# Autodesk Inventor assembly: unterArm
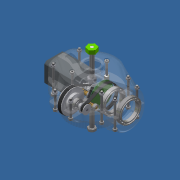
[picture p0: Inventor's stored thumbnail of the model, 180x180]
Saved by Autodesk Inventor 2016 (Build 200138000, 138)
## iProperties
Created: 2015-08-25
Part Number: unterArm
Material: Generisch
Document SubType Name: Assembly
Designer: 4ndreas
Mass: 1359.16 g
Surface Area: 1900.72 cm^2
Volume: 704.74 cm^3
Density: 1.92859 g/cm^3
Author: 4ndreas
## Documents named in this file (26)
- C:\Users\4ndreas\Documents\Inventor\RobotARM v2\v4\_assemblys\Forearm.iam
- C:\Users\4ndreas\Documents\Inventor\RobotARM v2\v4\forearm\Konstruktions-Assistent\Übertragung des Zahnriemens1.iam
- C:\Users\4ndreas\Documents\Inventor\RobotARM v2\v4\forearm\Konstruktions-Assistent\Übertragung des Zahnriemens2.iam
- C:\Users\4ndreas\Documents\Inventor\RobotARM v2\v4\_motors\Nema17_60.ipt
- C:\Users\4ndreas\Documents\Inventor\RobotARM v2\v4\_printed parts\unterArmSegment_A.ipt
- C:\Users\4ndreas\Documents\Inventor\RobotARM v2\v4\_printed parts\unterArmSegment_B.ipt
- C:\Users\4ndreas\Documents\Inventor\Content Center Files\R2014\de-DE\DIN BEARING(1)\DIN 625 SKF - SKF 61807.ipt
- C:\Users\4ndreas\Documents\Inventor\RobotARM v2\v4\forearm\Konstruktions-Assistent\Welle1.iam
- C:\Users\4ndreas\Documents\Inventor\Content Center Files\R2014\de-DE\DIN BEARING(1)\DIN 625 SKF - SKF 626.ipt
- C:\Users\4ndreas\Documents\Inventor\RobotARM v2\v4\_metal parts\Synchrone Riemenscheibe16.ipt
- C:\Users\4ndreas\Documents\Inventor\RobotARM v2\v4\_standard Parts\DIN 625 T1 - 619_6 - 6 x 11 x 5.ipt
- C:\Users\4ndreas\Documents\Inventor\RobotARM v2\v4\forearm\Konstruktions-Assistent\Welle2.iam
- C:\Users\4ndreas\Documents\Inventor\Content Center Files\R2014\de-DE\DIN 934\DIN 934 - M4 x 0,7.ipt
- C:\Users\4ndreas\Documents\Inventor\Content Center Files\R2014\de-DE\DIN 912\DIN 912 - M4 x 0,7 x 35 x 20.ipt
- C:\Users\4ndreas\Documents\Inventor\Content Center Files\R2014\de-DE\DIN 931-1\DIN 931-1 - M8 x 55.ipt
- C:\Users\4ndreas\Documents\Inventor\RobotARM v2\v4\_printed parts\Synchrone Riemenscheibe_60z_2.ipt
- C:\Users\4ndreas\Documents\Inventor\RobotARM v2\v4\_encoder\encoder_bare.ipt
- C:\Users\4ndreas\Documents\Inventor\RobotARM v2\v4\_encoder\EncoderMagnet.ipt
- C:\Users\4ndreas\Documents\Inventor\RobotARM v2\v4\_printed parts\magHexMount.ipt
- C:\Users\4ndreas\Documents\Inventor\RobotARM v2\v4\_standard Parts\DIN 912 - M4 x 0,7 x55.ipt
- C:\Users\4ndreas\Documents\Inventor\Content Center Files\R2014\de-DE\DIN 985\DIN 985 - M8.ipt
- C:\Users\4ndreas\Documents\Inventor\Content Center Files\R2014\de-DE\DIN 912\DIN 912 - M4 x 0,7 x 30 x 20.ipt
- C:\Users\4ndreas\Documents\Inventor\RobotARM v2\v4\_standard Parts\Distanzhuelse_M4x20mm.ipt
- C:\Users\4ndreas\Documents\Inventor\Content Center Files\R2014\de-DE\DIN 913\DIN 913 - M3 x 3.ipt
- C:\Users\4ndreas\Documents\Inventor\Content Center Files\R2014\de-DE\DIN 913\DIN 913 - M3 x 8.ipt
- C:\Users\4ndreas\Documents\Inventor\RobotARM v2\v4\_standard Parts\Distanzhuelse_M3x5mm.ipt
## Components (54 placed, 23 different names)
1. unterArmSegment_A:1 — Passend:12, Passend:28, Passend:30, Fluchtend:1, Passend:36, Passend:41, Passend:42, Passend:71, Passend:72, Passend:79, Passend:81, Passend:82, Passend:83, Passend:87, Passend:88, Passend:89, Passend:90, Passend:91, Passend:92, Passend:94, Passend:95, Passend:100, Passend:103, Passend:106, Passend:107, Passend:47, Passend:113, Winkel:2, Fluchtend:4, Passend:119, Passend:121, Passend:122, Passend:127, Passend:128, Passend:130, Passend:131, Passend:132, Passend:133, Passend:134, Passend:135, Passend:136, Passend:137, Passend:138, Passend:139
2. Nema17_60:1 — Fluchtend:2, Passend:32, Passend:33, Passend:39, Passend:41, Passend:42, Winkel:3
3. Übertragung des Zahnriemens:1 [sub-assembly] — Passend:27, Passend:40, Passend:112
4. Übertragung des Zahnriemens:2 [sub-assembly] — Passend:9, Passend:10, Passend:38
5. DIN 625 SKF SKF 61807:1 — Passend:9
6. DIN 625 SKF SKF 61807:2 — Passend:10, Passend:36
7. unterArmSegment_B:1 — Passend:12, Passend:28, Fluchtend:1, Passend:43, Passend:44, Passend:45, Passend:46, Passend:48, Passend:49, Passend:51, Passend:52, Passend:57, Passend:59, Passend:61, Passend:62, Passend:63, Passend:64, Passend:65, Passend:66, Passend:96, Passend:97, Passend:98, Passend:99, Passend:101, Passend:102, Passend:108, Fluchtend:5, Winkel:3, Passend:123, Passend:124, Passend:125, Passend:140, Passend:141, Passend:142, Passend:143
8. Welle:1 [sub-assembly] — Passend:16, Passend:17, Passend:27, Passend:37, Passend:109, Passend:129, Tangential:1, Tangential:2, Tangential:3
9. DIN 625 SKF SKF 626:2 — Passend:16, Passend:30
10. DIN 625 SKF SKF 626:1 — Passend:17, Passend:51, Passend:110
11. Synchrone Riemenscheibe1:1 — Passend:37, Passend:38, Passend:129, Passend:144, Passend:145
12. Synchrone Riemenscheibe1:2 — Passend:39, Passend:40, Passend:146, Passend:147
13. DIN 625 - T1 619/6 - 6 x 15 x 5:1 — Passend:45, Passend:47
14. DIN 625 - T1 619/6 - 6 x 15 x 5:2 — Passend:43, Passend:49
15. DIN 625 - T1 619/6 - 6 x 15 x 5:3 — Passend:44, Passend:52, Passend:53, Passend:54
16. DIN 625 - T1 619/6 - 6 x 15 x 5:4 — Passend:46, Passend:48, Passend:55, Passend:56
17. Welle:2 [sub-assembly] — Passend:53, Passend:54
18. Welle:3 [sub-assembly] — Passend:55, Passend:56
19. DIN 912 - ersetzt durch DIN EN ISO 4762 M4 x 55:1 — Passend:57, Passend:59, Passend:75
20. DIN 912 - ersetzt durch DIN EN ISO 4762 M4 x 55:1 — Passend:61, Passend:64, Passend:77, Passend:93
21. DIN 912 - ersetzt durch DIN EN ISO 4762 M4 x 55:1 — Passend:62, Passend:63, Passend:73
22. DIN 912 - ersetzt durch DIN EN ISO 4762 M4 x 55:1 — Passend:65, Passend:66, Passend:78
23. DIN 912 - ersetzt durch DIN EN ISO 4762 M4 x 35:1 — Passend:96, Passend:98
24. DIN 912 - ersetzt durch DIN EN ISO 4762 M4 x 35:2 — Passend:97, Passend:99
25. DIN 912 - ersetzt durch DIN EN ISO 4762 M4 x 55:1 — Passend:119, Passend:120, Passend:123
26. DIN 912 - ersetzt durch DIN EN ISO 4762 M4 x 55:2 — Passend:124, Passend:125, Passend:126
27. DIN 934 - ersetzt durch DIN EN 24032/28673/28674 M4:1 — Passend:72, Passend:89, Passend:90
28. DIN 934 - ersetzt durch DIN EN 24032/28673/28674 M4:2 — Passend:73, Passend:91, Passend:92
29. DIN 934 - ersetzt durch DIN EN 24032/28673/28674 M4:3 — Passend:71, Passend:87, Passend:88
30. DIN 934 - ersetzt durch DIN EN 24032/28673/28674 M4:4 — Passend:75, Passend:81, Passend:82
31. DIN 934 - ersetzt durch DIN EN 24032/28673/28674 M4:6 — Passend:77, Passend:93, Passend:94, Passend:95
32. DIN 934 - ersetzt durch DIN EN 24032/28673/28674 M4:8 — Passend:78, Passend:79, Passend:83
33. DIN 931-1 - ersetzt durch DIN EN 24014 M8 x 55:1 — Passend:100, Passend:103, Passend:104, Passend:116, Passend:117, Passend:118
34. DIN 931-1 - ersetzt durch DIN EN 24014 M8 x 55:2 — Passend:101, Passend:102, Passend:105
35. DIN 985 - ersetzt durch DIN EN ISO 10511 M8:1 — Passend:104, Fluchtend:3, Passend:106, Passend:107
36. DIN 985 - ersetzt durch DIN EN ISO 10511 M8:2 — Passend:105, Fluchtend:3, Passend:108
37. Synchrone Riemenscheibe2:1 — Passend:109, Passend:110, Passend:149, Passend:150, Passend:151
38. encoder_bare:1 — Passend:111, Passend:113, Winkel:2, Fluchtend:4, Fluchtend:5
39. EncoderMagnet:1 — Passend:114, Passend:115
40. magHexMount:1 — Passend:114, Passend:115, Passend:116, Passend:117, Passend:118
41. DIN 934 - ersetzt durch DIN EN 24032/28673/28674 M4:9 — Passend:120, Passend:121, Passend:122
42. DIN 934 - ersetzt durch DIN EN 24032/28673/28674 M4:10 — Passend:126, Passend:127, Passend:128
43. Distanzhuelse_M4x20mm:1 — Passend:131, Passend:133, Passend:134
44. Distanzhuelse_M4x20mm:2 — Passend:130, Passend:132, Passend:135
45. DIN 912 - ersetzt durch DIN EN ISO 4762 M4 x 30:1 — Passend:137, Passend:138
46. DIN 912 - ersetzt durch DIN EN ISO 4762 M4 x 30:2 — Passend:136, Passend:139
47. DIN 912 - ersetzt durch DIN EN ISO 4762 M4 x 30:3 — Passend:140, Passend:142
48. DIN 912 - ersetzt durch DIN EN ISO 4762 M4 x 30:4 — Passend:141, Passend:143
49. DIN 913 M3 x 3:1 — Tangential:2, Passend:145
50. DIN 913 M3 x 3:2 — Tangential:1, Passend:144
51. DIN 913 M3 x 3:3 — Passend:147
52. DIN 913 M3 x 3:4 — Passend:146
53. DIN 913 M3 x 8:1 — Passend:148, Passend:149, Tangential:3
54. Distanzhuelse_M3x5mm:1 — Passend:148, Passend:150, Passend:151
## Relationships (123: Mate 113, Flush 5, Tangent 3, Angle 2)
- Passend:9 [Mate]: Übertragung des Zahnriemens:2 ↔ DIN 625 SKF SKF 61807:1
- Passend:10 [Mate]: Übertragung des Zahnriemens:2 ↔ DIN 625 SKF SKF 61807:2
- Passend:12 [Mate]: unterArmSegment_A:1 ↔ unterArmSegment_B:1
- Passend:16 [Mate]: Welle:1 ↔ DIN 625 SKF SKF 626:2
- Passend:17 [Mate]: Welle:1 ↔ DIN 625 SKF SKF 626:1
- Passend:27 [Mate]: Übertragung des Zahnriemens:1 ↔ Welle:1
- Passend:28 [Mate]: unterArmSegment_A:1 ↔ unterArmSegment_B:1
- Passend:30 [Mate]: unterArmSegment_A:1 ↔ DIN 625 SKF SKF 626:2
- Fluchtend:1 [Flush]: unterArmSegment_A:1 ↔ unterArmSegment_B:1
- Fluchtend:2 [Flush]: Nema17_60:1
- Passend:32 [Mate]: Nema17_60:1
- Passend:33 [Mate]: Nema17_60:1
- Passend:36 [Mate]: unterArmSegment_A:1 ↔ DIN 625 SKF SKF 61807:2
- Passend:37 [Mate]: Welle:1 ↔ Synchrone Riemenscheibe1:1
- Passend:38 [Mate] (0.25 mm): Übertragung des Zahnriemens:2 ↔ Synchrone Riemenscheibe1:1
- Passend:39 [Mate]: Nema17_60:1 ↔ Synchrone Riemenscheibe1:2
- Passend:40 [Mate] (0.25 mm): Übertragung des Zahnriemens:1 ↔ Synchrone Riemenscheibe1:2
- Passend:41 [Mate]: unterArmSegment_A:1 ↔ Nema17_60:1
- Passend:42 [Mate]: unterArmSegment_A:1 ↔ Nema17_60:1
- Passend:43 [Mate]: unterArmSegment_B:1 ↔ DIN 625 - T1 619/6 - 6 x 15 x 5:2
- Passend:44 [Mate]: unterArmSegment_B:1 ↔ DIN 625 - T1 619/6 - 6 x 15 x 5:3
- Passend:45 [Mate]: unterArmSegment_B:1 ↔ DIN 625 - T1 619/6 - 6 x 15 x 5:1
- Passend:46 [Mate]: unterArmSegment_B:1 ↔ DIN 625 - T1 619/6 - 6 x 15 x 5:4
- Passend:47 [Mate]: unterArmSegment_A:1 ↔ DIN 625 - T1 619/6 - 6 x 15 x 5:1
- Passend:48 [Mate]: unterArmSegment_B:1 ↔ DIN 625 - T1 619/6 - 6 x 15 x 5:4
- Passend:49 [Mate]: unterArmSegment_B:1 ↔ DIN 625 - T1 619/6 - 6 x 15 x 5:2
- Passend:51 [Mate]: unterArmSegment_B:1 ↔ DIN 625 SKF SKF 626:1
- Passend:52 [Mate]: unterArmSegment_B:1 ↔ DIN 625 - T1 619/6 - 6 x 15 x 5:3
- Passend:53 [Mate]: DIN 625 - T1 619/6 - 6 x 15 x 5:3 ↔ Welle:2
- Passend:54 [Mate]: DIN 625 - T1 619/6 - 6 x 15 x 5:3 ↔ Welle:2
- Passend:55 [Mate]: DIN 625 - T1 619/6 - 6 x 15 x 5:4 ↔ Welle:3
- Passend:56 [Mate]: DIN 625 - T1 619/6 - 6 x 15 x 5:4 ↔ Welle:3
- Passend:57 [Mate]: unterArmSegment_B:1 ↔ DIN 912 - ersetzt durch DIN EN ISO 4762 M4 x 55:1
- Passend:59 [Mate]: unterArmSegment_B:1 ↔ DIN 912 - ersetzt durch DIN EN ISO 4762 M4 x 55:1
- Passend:61 [Mate]: unterArmSegment_B:1 ↔ DIN 912 - ersetzt durch DIN EN ISO 4762 M4 x 55:1
- Passend:62 [Mate]: unterArmSegment_B:1 ↔ DIN 912 - ersetzt durch DIN EN ISO 4762 M4 x 55:1
- Passend:63 [Mate]: unterArmSegment_B:1 ↔ DIN 912 - ersetzt durch DIN EN ISO 4762 M4 x 55:1
- Passend:64 [Mate]: unterArmSegment_B:1 ↔ DIN 912 - ersetzt durch DIN EN ISO 4762 M4 x 55:1
- Passend:65 [Mate]: unterArmSegment_B:1 ↔ DIN 912 - ersetzt durch DIN EN ISO 4762 M4 x 55:1
- Passend:66 [Mate]: unterArmSegment_B:1 ↔ DIN 912 - ersetzt durch DIN EN ISO 4762 M4 x 55:1
- Passend:71 [Mate]: unterArmSegment_A:1 ↔ DIN 934 - ersetzt durch DIN EN 24032/28673/28674 M4:3
- Passend:72 [Mate]: unterArmSegment_A:1 ↔ DIN 934 - ersetzt durch DIN EN 24032/28673/28674 M4:1
- Passend:73 [Mate]: DIN 912 - ersetzt durch DIN EN ISO 4762 M4 x 55:1 ↔ DIN 934 - ersetzt durch DIN EN 24032/28673/28674 M4:2
- Passend:75 [Mate]: DIN 912 - ersetzt durch DIN EN ISO 4762 M4 x 55:1 ↔ DIN 934 - ersetzt durch DIN EN 24032/28673/28674 M4:4
- Passend:77 [Mate]: DIN 912 - ersetzt durch DIN EN ISO 4762 M4 x 55:1 ↔ DIN 934 - ersetzt durch DIN EN 24032/28673/28674 M4:6
- Passend:78 [Mate]: DIN 912 - ersetzt durch DIN EN ISO 4762 M4 x 55:1 ↔ DIN 934 - ersetzt durch DIN EN 24032/28673/28674 M4:8
- Passend:79 [Mate]: unterArmSegment_A:1 ↔ DIN 934 - ersetzt durch DIN EN 24032/28673/28674 M4:8
- Passend:81 [Mate]: unterArmSegment_A:1 ↔ DIN 934 - ersetzt durch DIN EN 24032/28673/28674 M4:4
- Passend:82 [Mate]: unterArmSegment_A:1 ↔ DIN 934 - ersetzt durch DIN EN 24032/28673/28674 M4:4
- Passend:83 [Mate]: unterArmSegment_A:1 ↔ DIN 934 - ersetzt durch DIN EN 24032/28673/28674 M4:8
- Passend:87 [Mate]: unterArmSegment_A:1 ↔ DIN 934 - ersetzt durch DIN EN 24032/28673/28674 M4:3
- Passend:88 [Mate]: unterArmSegment_A:1 ↔ DIN 934 - ersetzt durch DIN EN 24032/28673/28674 M4:3
- Passend:89 [Mate]: unterArmSegment_A:1 ↔ DIN 934 - ersetzt durch DIN EN 24032/28673/28674 M4:1
- Passend:90 [Mate]: unterArmSegment_A:1 ↔ DIN 934 - ersetzt durch DIN EN 24032/28673/28674 M4:1
- Passend:91 [Mate]: unterArmSegment_A:1 ↔ DIN 934 - ersetzt durch DIN EN 24032/28673/28674 M4:2
- Passend:92 [Mate]: unterArmSegment_A:1 ↔ DIN 934 - ersetzt durch DIN EN 24032/28673/28674 M4:2
- Passend:93 [Mate]: DIN 912 - ersetzt durch DIN EN ISO 4762 M4 x 55:1 ↔ DIN 934 - ersetzt durch DIN EN 24032/28673/28674 M4:6
- Passend:94 [Mate]: unterArmSegment_A:1 ↔ DIN 934 - ersetzt durch DIN EN 24032/28673/28674 M4:6
- Passend:95 [Mate]: unterArmSegment_A:1 ↔ DIN 934 - ersetzt durch DIN EN 24032/28673/28674 M4:6
- Passend:96 [Mate]: unterArmSegment_B:1 ↔ DIN 912 - ersetzt durch DIN EN ISO 4762 M4 x 35:1
- Passend:97 [Mate]: unterArmSegment_B:1 ↔ DIN 912 - ersetzt durch DIN EN ISO 4762 M4 x 35:2
- Passend:98 [Mate]: unterArmSegment_B:1 ↔ DIN 912 - ersetzt durch DIN EN ISO 4762 M4 x 35:1
- Passend:99 [Mate]: unterArmSegment_B:1 ↔ DIN 912 - ersetzt durch DIN EN ISO 4762 M4 x 35:2
- Passend:100 [Mate]: unterArmSegment_A:1 ↔ DIN 931-1 - ersetzt durch DIN EN 24014 M8 x 55:1
- Passend:101 [Mate]: unterArmSegment_B:1 ↔ DIN 931-1 - ersetzt durch DIN EN 24014 M8 x 55:2
- Passend:102 [Mate] (28 mm): unterArmSegment_B:1 ↔ DIN 931-1 - ersetzt durch DIN EN 24014 M8 x 55:2
- Passend:103 [Mate] (29 mm): unterArmSegment_A:1 ↔ DIN 931-1 - ersetzt durch DIN EN 24014 M8 x 55:1
- Passend:104 [Mate]: DIN 931-1 - ersetzt durch DIN EN 24014 M8 x 55:1 ↔ DIN 985 - ersetzt durch DIN EN ISO 10511 M8:1
- Passend:105 [Mate]: DIN 931-1 - ersetzt durch DIN EN 24014 M8 x 55:2 ↔ DIN 985 - ersetzt durch DIN EN ISO 10511 M8:2
- Fluchtend:3 [Flush]: DIN 985 - ersetzt durch DIN EN ISO 10511 M8:1 ↔ DIN 985 - ersetzt durch DIN EN ISO 10511 M8:2
- Passend:106 [Mate]: unterArmSegment_A:1 ↔ DIN 985 - ersetzt durch DIN EN ISO 10511 M8:1
- Passend:107 [Mate]: unterArmSegment_A:1 ↔ DIN 985 - ersetzt durch DIN EN ISO 10511 M8:1
- Passend:108 [Mate]: unterArmSegment_B:1 ↔ DIN 985 - ersetzt durch DIN EN ISO 10511 M8:2
- Passend:109 [Mate]: Welle:1 ↔ Synchrone Riemenscheibe2:1
- Passend:110 [Mate]: DIN 625 SKF SKF 626:1 ↔ Synchrone Riemenscheibe2:1
- Passend:111 [Mate]: encoder_bare:1
- Passend:112 [Mate]: Übertragung des Zahnriemens:1
- Passend:113 [Mate]: unterArmSegment_A:1 ↔ encoder_bare:1
- Winkel:2 [Angle] (15 deg): unterArmSegment_A:1 ↔ encoder_bare:1
- Fluchtend:4 [Flush]: unterArmSegment_A:1 ↔ encoder_bare:1
- Fluchtend:5 [Flush]: unterArmSegment_B:1 ↔ encoder_bare:1
- Winkel:3 [Angle] (0 deg): Nema17_60:1 ↔ unterArmSegment_B:1
- Passend:114 [Mate]: EncoderMagnet:1 ↔ magHexMount:1
- Passend:115 [Mate]: EncoderMagnet:1 ↔ magHexMount:1
- Passend:116 [Mate]: DIN 931-1 - ersetzt durch DIN EN 24014 M8 x 55:1 ↔ magHexMount:1
- Passend:117 [Mate]: DIN 931-1 - ersetzt durch DIN EN 24014 M8 x 55:1 ↔ magHexMount:1
- Passend:118 [Mate]: DIN 931-1 - ersetzt durch DIN EN 24014 M8 x 55:1 ↔ magHexMount:1
- Passend:119 [Mate]: unterArmSegment_A:1 ↔ DIN 912 - ersetzt durch DIN EN ISO 4762 M4 x 55:1
- Passend:120 [Mate]: DIN 912 - ersetzt durch DIN EN ISO 4762 M4 x 55:1 ↔ DIN 934 - ersetzt durch DIN EN 24032/28673/28674 M4:9
- Passend:121 [Mate]: unterArmSegment_A:1 ↔ DIN 934 - ersetzt durch DIN EN 24032/28673/28674 M4:9
- Passend:122 [Mate]: unterArmSegment_A:1 ↔ DIN 934 - ersetzt durch DIN EN 24032/28673/28674 M4:9
- Passend:123 [Mate]: unterArmSegment_B:1 ↔ DIN 912 - ersetzt durch DIN EN ISO 4762 M4 x 55:1
- Passend:124 [Mate]: unterArmSegment_B:1 ↔ DIN 912 - ersetzt durch DIN EN ISO 4762 M4 x 55:2
- Passend:125 [Mate]: unterArmSegment_B:1 ↔ DIN 912 - ersetzt durch DIN EN ISO 4762 M4 x 55:2
- Passend:126 [Mate]: DIN 912 - ersetzt durch DIN EN ISO 4762 M4 x 55:2 ↔ DIN 934 - ersetzt durch DIN EN 24032/28673/28674 M4:10
- Passend:127 [Mate]: unterArmSegment_A:1 ↔ DIN 934 - ersetzt durch DIN EN 24032/28673/28674 M4:10
- Passend:128 [Mate]: unterArmSegment_A:1 ↔ DIN 934 - ersetzt durch DIN EN 24032/28673/28674 M4:10
- Passend:129 [Mate]: Welle:1 ↔ Synchrone Riemenscheibe1:1
- Passend:130 [Mate]: unterArmSegment_A:1 ↔ Distanzhuelse_M4x20mm:2
- Passend:131 [Mate]: unterArmSegment_A:1 ↔ Distanzhuelse_M4x20mm:1
- Passend:132 [Mate]: unterArmSegment_A:1 ↔ Distanzhuelse_M4x20mm:2
- Passend:133 [Mate]: unterArmSegment_A:1 ↔ Distanzhuelse_M4x20mm:1
- Passend:134 [Mate]: unterArmSegment_A:1 ↔ Distanzhuelse_M4x20mm:1
- Passend:135 [Mate]: unterArmSegment_A:1 ↔ Distanzhuelse_M4x20mm:2
- Passend:136 [Mate]: unterArmSegment_A:1 ↔ DIN 912 - ersetzt durch DIN EN ISO 4762 M4 x 30:2
- Passend:137 [Mate]: unterArmSegment_A:1 ↔ DIN 912 - ersetzt durch DIN EN ISO 4762 M4 x 30:1
- Passend:138 [Mate]: unterArmSegment_A:1 ↔ DIN 912 - ersetzt durch DIN EN ISO 4762 M4 x 30:1
- Passend:139 [Mate]: unterArmSegment_A:1 ↔ DIN 912 - ersetzt durch DIN EN ISO 4762 M4 x 30:2
- Passend:140 [Mate]: unterArmSegment_B:1 ↔ DIN 912 - ersetzt durch DIN EN ISO 4762 M4 x 30:3
- Passend:141 [Mate]: unterArmSegment_B:1 ↔ DIN 912 - ersetzt durch DIN EN ISO 4762 M4 x 30:4
- Passend:142 [Mate]: unterArmSegment_B:1 ↔ DIN 912 - ersetzt durch DIN EN ISO 4762 M4 x 30:3
- Passend:143 [Mate]: unterArmSegment_B:1 ↔ DIN 912 - ersetzt durch DIN EN ISO 4762 M4 x 30:4
- Tangential:1: Welle:1 ↔ DIN 913 M3 x 3:2
- Tangential:2: Welle:1 ↔ DIN 913 M3 x 3:1
- Passend:144 [Mate]: Synchrone Riemenscheibe1:1 ↔ DIN 913 M3 x 3:2
- Passend:145 [Mate]: Synchrone Riemenscheibe1:1 ↔ DIN 913 M3 x 3:1
- Passend:146 [Mate]: Synchrone Riemenscheibe1:2 ↔ DIN 913 M3 x 3:4
- Passend:147 [Mate]: Synchrone Riemenscheibe1:2 ↔ DIN 913 M3 x 3:3
- Passend:148 [Mate]: DIN 913 M3 x 8:1 ↔ Distanzhuelse_M3x5mm:1
- Passend:149 [Mate]: Synchrone Riemenscheibe2:1 ↔ DIN 913 M3 x 8:1
- Passend:150 [Mate]: Synchrone Riemenscheibe2:1 ↔ Distanzhuelse_M3x5mm:1
- Passend:151 [Mate]: Synchrone Riemenscheibe2:1 ↔ Distanzhuelse_M3x5mm:1
- Tangential:3: Welle:1 ↔ DIN 913 M3 x 8:1
